# Autodesk Inventor assembly: tip_3_ass_base
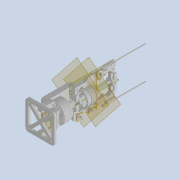
[picture p0: Inventor's stored thumbnail of the model, 180x180]
Saved by Autodesk Inventor 2020 (Build 240168000, 168)
## iProperties
Created: 2021-09-09
Part Number: tip_3_ass_base
Document SubType Name: Assembly
Designer: Shuang Peng
Author: Shuang Peng
## Documents named in this file (12)
- D:\projects-3\torque fb tip\hardware\tip_3\tip_3_ass_base.iam
- D:\projects-3\torque fb tip\hardware\tip_3\pin_3_30.ipt
- D:\projects-3\torque fb tip\hardware\tip_3\bearing_3_6_2.ipt
- D:\projects-3\torque fb tip\hardware\tip_3\bearing_hh_1.ipt
- D:\projects-3\torque fb tip\hardware\tip_3\c_roller_1.ipt
- D:\projects-3\torque fb tip\hardware\tip_3\bw_ass_1.iam
- D:\projects-3\torque fb tip\hardware\tip_3\ext_shell_2.ipt
- D:\projects-3\torque fb tip\hardware\tip_3\roller_4.ipt
- D:\projects-3\torque fb tip\hardware\tip_3\mot_27_ass.iam
- D:\projects-3\torque fb tip\hardware\tip_3\mot_trans_1.ipt
- D:\projects-3\torque fb tip\hardware\tip_3\mot_test_enc_hh_1.ipt
- D:\projects-3\torque fb tip\hardware\tip_3\base_stand_1.ipt
## Components (21 placed, 11 different names)
1. pin_3_30:1 — Insert:18
2. pin_3_30:2 — Insert:25
3. bearing_3_6_2:1 — Flush:1, Insert:15, Insert:25
4. bearing_hh_1:1 — Flush:1, Flush:3, Insert:15, Insert:21
5. bearing_3_6_2:2 — Insert:6, Insert:18, Insert:30
6. bearing_hh_1:2 — Insert:6, Flush:3, Insert:19, Insert:20
7. bearing_3_6_2:3 — Insert:11, Insert:23
8. bearing_3_6_2:4 — Flush:7, Insert:10, Insert:24
9. c_roller_1:1 — Flush:7, Insert:10
10. c_roller_1:2 — Insert:11
11. bearing_3_6_2:5 — Insert:22
12. c_roller_1:3
13. bw_ass_1:1 [sub-assembly] — Insert:26, Insert:27
14. bw_ass_1:2 [sub-assembly] — Insert:28, Insert:29
15. ext_shell_2:1 — Insert:19, Insert:20, Insert:21, Insert:22, Insert:23, Insert:24, Insert:26, Insert:27, Insert:28, Insert:29, Insert:34, Angle:1, Insert:35, Insert:36
16. roller_4:1 — Insert:31
17. roller_4:2 — Insert:30, Insert:31
18. mot_27_ass:1 [sub-assembly] — Flush:8, Insert:32, Insert:33, Angle:1
19. mot_trans_1:1 — Flush:8, Insert:32, Insert:33, Insert:34
20. mot_test_enc_hh_1:1 — Insert:35, Insert:36, Flush:9, Flush:10, Flush:11, Insert:37
21. base_stand_1:1 — Flush:9, Flush:10, Flush:11, Insert:37
## Relationships (34: Insert 25, Flush 8, Angle 1)
- Flush:1: bearing_3_6_2:1 ↔ bearing_hh_1:1
- [Flush]: bearing_3_6_2:2 ↔ bearing_hh_1:2
- Insert:6: bearing_3_6_2:2 ↔ bearing_hh_1:2
- Flush:3: bearing_hh_1:1 ↔ bearing_hh_1:2
- Flush:7: bearing_3_6_2:4 ↔ c_roller_1:1
- Insert:10: bearing_3_6_2:4 ↔ c_roller_1:1
- Insert:11: bearing_3_6_2:3 ↔ c_roller_1:2
- [Insert]: bearing_3_6_2:5 ↔ c_roller_1:3
- Insert:15: bearing_3_6_2:1 ↔ bearing_hh_1:1
- Insert:18 (-15 mm): pin_3_30:1 ↔ bearing_3_6_2:2
- Insert:19: bearing_hh_1:2 ↔ ext_shell_2:1
- Insert:20: bearing_hh_1:2 ↔ ext_shell_2:1
- Insert:21: bearing_hh_1:1 ↔ ext_shell_2:1
- Insert:22: bearing_3_6_2:5 ↔ ext_shell_2:1
- Insert:23: bearing_3_6_2:3 ↔ ext_shell_2:1
- Insert:24: bearing_3_6_2:4 ↔ ext_shell_2:1
- Insert:25 (-20 mm): pin_3_30:2 ↔ bearing_3_6_2:1
- Insert:26: bw_ass_1:1 ↔ ext_shell_2:1
- Insert:27: bw_ass_1:1 ↔ ext_shell_2:1
- Insert:28: bw_ass_1:2 ↔ ext_shell_2:1
- Insert:29: bw_ass_1:2 ↔ ext_shell_2:1
- Insert:30: bearing_3_6_2:2 ↔ roller_4:2
- Insert:31: roller_4:1 ↔ roller_4:2
- Flush:8: mot_27_ass:1 ↔ mot_trans_1:1
- Insert:32: mot_27_ass:1 ↔ mot_trans_1:1
- Insert:33: mot_27_ass:1 ↔ mot_trans_1:1
- Insert:34 (1 mm): ext_shell_2:1 ↔ mot_trans_1:1
- Angle:1 (45 deg): ext_shell_2:1 ↔ mot_27_ass:1
- Insert:35: ext_shell_2:1 ↔ mot_test_enc_hh_1:1
- Insert:36: ext_shell_2:1 ↔ mot_test_enc_hh_1:1
- Flush:9: mot_test_enc_hh_1:1 ↔ base_stand_1:1
- Flush:10 (10 mm): mot_test_enc_hh_1:1 ↔ base_stand_1:1
- Flush:11: mot_test_enc_hh_1:1 ↔ base_stand_1:1
- Insert:37: mot_test_enc_hh_1:1 ↔ base_stand_1:1
## Named parameters: d5_d4 = 0 mm, d19_d18 = 0 mm
